# Autodesk Inventor assembly: Piston Wall Guide Wide assy
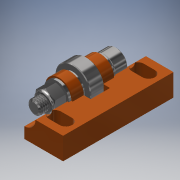
[picture p0: Inventor's stored thumbnail of the model, 180x180]
Saved by Autodesk Inventor 2018 (Build 220112000, 112)
## iProperties
Created: 2017-09-27
Part Number: Piston Wall Guide Wide assy
Document SubType Name: Assembly
Designer: Gabriel Smolnycki
Author: Gabriel Smolnycki
## Documents named in this file (6)
- H:\dev\planb\mechanics\V1INV\Subassemblies\Piston Wall Guide Wide assy.iam
- H:\dev\planb\mechanics\V1INV\Piston\Piston Wall Guide Wide.ipt
- H:\dev\planb\mechanics\V1INV\Hardware\4x13 SS Ball Bearing (7804K103).ipt
- H:\dev\planb\mechanics\V1INV\Hardware\M4 SS Locknut.ipt
- H:\dev\planb\mechanics\V1INV\Hardware\M4 SS Washer.ipt
- H:\dev\planb\mechanics\V1INV\Hardware\M4x25 SS SHCS.ipt
## Components (8 placed, 5 different names)
1. Piston Wall Guide Wide:1 — Mate:1, Insert:1, Insert:2, Insert:3, Insert:4
2. 4x13 SS Ball Bearing (7804K103):1 — Mate:1, Insert:5
3. M4 SS Locknut:1 — Insert:6
4. M4 SS Washer:1 — Insert:1, Insert:5
5. M4 SS Washer:2 — Insert:2
6. M4 SS Washer:3 — Insert:4, Insert:7
7. M4 SS Washer:4 — Insert:3, Insert:6
8. M4x25 SS SHCS:1 — Insert:7
## Relationships (8: Insert 7, Mate 1)
- Mate:1: Piston Wall Guide Wide:1 ↔ 4x13 SS Ball Bearing (7804K103):1
- Insert:1: Piston Wall Guide Wide:1 ↔ M4 SS Washer:1
- Insert:2: Piston Wall Guide Wide:1 ↔ M4 SS Washer:2
- Insert:3: Piston Wall Guide Wide:1 ↔ M4 SS Washer:4
- Insert:4: Piston Wall Guide Wide:1 ↔ M4 SS Washer:3
- Insert:5: 4x13 SS Ball Bearing (7804K103):1 ↔ M4 SS Washer:1
- Insert:6: M4 SS Locknut:1 ↔ M4 SS Washer:4
- Insert:7: M4 SS Washer:3 ↔ M4x25 SS SHCS:1
